# Autodesk Inventor assembly: Ensamble Mecanismo cilindro
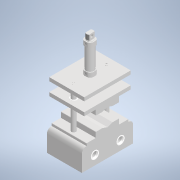
[picture p0: Inventor's stored thumbnail of the model, 180x180]
Saved by Autodesk Inventor 2021 (Build 250183000, 183)
## iProperties
Created: 2020-01-15
Part Number: Ensamble Mecanismo cilindro
Document SubType Name: Assembly
Designer: Nelson
Sending System: SolidWorks 2020
Last Author: Micro
Last Saved: 2020-01-16
Author: Nelson
## Documents named in this file (9)
- D:\Nelson\Documentos\Inventor\PrensaHidraulica_Automatizada\Ensamble Mecanismo cilindro.iam
- Ensamble mecanismo cilindro.iam
- D:\Nelson\Documentos\Inventor\PrensaHidraulica_Automatizada\Base soporte tubos.ipt
- D:\Nelson\Documentos\Inventor\PrensaHidraulica_Automatizada\Buje de base soporte.ipt
- D:\Nelson\Documentos\Inventor\PrensaHidraulica_Automatizada\Eje roscado base soporte tubo.ipt
- D:\Nelson\Documentos\Inventor\PrensaHidraulica_Automatizada\193992 DSNU-32-60-PPS-A---(60PPSA---00--0-------0).iam
- D:\Nelson\Documentos\Inventor\PrensaHidraulica_Automatizada\Soporte Piston.ipt
- D:\Nelson\Documentos\Inventor\PrensaHidraulica_Automatizada\Soporte Superior Tubos.ipt
- D:\Nelson\Documentos\Inventor\PrensaHidraulica_Automatizada\Buje soporte superior.ipt
## Components (14 placed, 7 different names)
1. Base soporte tubos:1 — Mate:7, Mate:8, Mate:9, Mate:10, Mate:11, Mate:12, Mate:13, Mate:14, Mate:27, Mate:28, Mate:29, Mate:30
2. Buje de base soporte:1 — Mate:7, Mate:8
3. Buje de base soporte:2 — Mate:9, Mate:10
4. Buje de base soporte:3 — Mate:11, Mate:12
5. Buje de base soporte:4 — Mate:13, Mate:14
6. Eje roscado base soporte tubo:1 — Mate:27, Mate:28, Mate:31, Mate:33, Mate:45
7. Eje roscado base soporte tubo:2 — Mate:29, Mate:30, Mate:32, Mate:44
8. 193992 DSNU-32-60-PPS-A---(60PPSA---00--0-------0):1 [sub-assembly] — Mate:34, Mate:35, Mate:46
9. Soporte Piston:1 — Mate:31, Mate:32, Mate:33, Mate:34, Mate:35
10. Soporte Superior Tubos:1 — Mate:36, Mate:37, Mate:38, Mate:39, Mate:40, Mate:41, Mate:42, Mate:43, Mate:46
11. Buje soporte superior:1 — Mate:38, Mate:39, Mate:44
12. Buje soporte superior:2 — Mate:36, Mate:37, Mate:45
13. Buje soporte superior:3 — Mate:40, Mate:41
14. Buje soporte superior:4 — Mate:42, Mate:43
## Relationships (28: Mate 28)
- Mate:7: Base soporte tubos:1 ↔ Buje de base soporte:1
- Mate:8: Base soporte tubos:1 ↔ Buje de base soporte:1
- Mate:9: Base soporte tubos:1 ↔ Buje de base soporte:2
- Mate:10: Base soporte tubos:1 ↔ Buje de base soporte:2
- Mate:11: Base soporte tubos:1 ↔ Buje de base soporte:3
- Mate:12: Base soporte tubos:1 ↔ Buje de base soporte:3
- Mate:13: Base soporte tubos:1 ↔ Buje de base soporte:4
- Mate:14: Base soporte tubos:1 ↔ Buje de base soporte:4
- Mate:27: Base soporte tubos:1 ↔ Eje roscado base soporte tubo:1
- Mate:28: Base soporte tubos:1 ↔ Eje roscado base soporte tubo:1
- Mate:29: Base soporte tubos:1 ↔ Eje roscado base soporte tubo:2
- Mate:30: Base soporte tubos:1 ↔ Eje roscado base soporte tubo:2
- Mate:31: Eje roscado base soporte tubo:1 ↔ Soporte Piston:1
- Mate:32: Eje roscado base soporte tubo:2 ↔ Soporte Piston:1
- Mate:33: Eje roscado base soporte tubo:1 ↔ Soporte Piston:1
- Mate:34: 193992 DSNU-32-60-PPS-A---(60PPSA---00--0-------0):1 ↔ Soporte Piston:1
- Mate:35: 193992 DSNU-32-60-PPS-A---(60PPSA---00--0-------0):1 ↔ Soporte Piston:1
- Mate:36: Soporte Superior Tubos:1 ↔ Buje soporte superior:2
- Mate:37: Soporte Superior Tubos:1 ↔ Buje soporte superior:2
- Mate:38: Soporte Superior Tubos:1 ↔ Buje soporte superior:1
- Mate:39: Soporte Superior Tubos:1 ↔ Buje soporte superior:1
- Mate:40: Soporte Superior Tubos:1 ↔ Buje soporte superior:3
- Mate:41: Soporte Superior Tubos:1 ↔ Buje soporte superior:3
- Mate:42: Soporte Superior Tubos:1 ↔ Buje soporte superior:4
- Mate:43: Soporte Superior Tubos:1 ↔ Buje soporte superior:4
- Mate:44: Eje roscado base soporte tubo:2 ↔ Buje soporte superior:1
- Mate:45: Eje roscado base soporte tubo:1 ↔ Buje soporte superior:2
- Mate:46: 193992 DSNU-32-60-PPS-A---(60PPSA---00--0-------0):1 ↔ Soporte Superior Tubos:1
